# Autodesk Inventor assembly: Remote Bottom Print Assembly
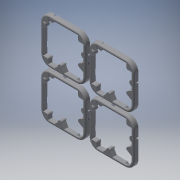
[picture p0: Inventor's stored thumbnail of the model, 180x180]
Saved by Autodesk Inventor 2018 (Build 220112000, 112)
## iProperties
Created: 2015-10-15
Part Number: Remote Bottom Print Assembly
Document SubType Name: Assembly
Designer: Sam Clay
Author: Sam Clay
## Documents named in this file (2)
- Z:\enclosure\inventor\Remote Bottom Print Assembly.iam
- Z:\enclosure\inventor\Remote Bottom.ipt
## Components (4 placed, 1 different names)
1. Remote Bottom:1
2. Remote Bottom:2
3. Remote Bottom:3
4. Remote Bottom:4
## Component patterns: (4 elements, first: Remote Bottom:1)
